# Autodesk Inventor assembly: 3_8 Shawny Lift 40t Idler
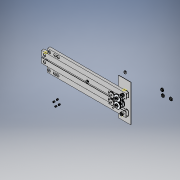
[picture p0: Inventor's stored thumbnail of the model, 180x180]
Saved by Autodesk Inventor 2018 (Build 220112000, 112)
## iProperties
Created: 2019-01-14
Part Number: 3_8 Shawny Lift 40t Idler
Document SubType Name: Assembly
Designer: Gabriel
Author: Gabriel
## Documents named in this file (10)
- C:\Users\Gabriel\Documents\3_8 Shawny Lift 40t Idler.iam
- C:\Users\Gabriel\Documents\8T spur gear 775.ipt
- C:\Users\Gabriel\Documents\36in Aluminum Channel OG.ipt
- C:\Users\Gabriel\Documents\Sanded Hex Rod.ipt
- C:\Users\Gabriel\Documents\Spacer 1 16 in.ipt
- C:\Users\Gabriel\Documents\Flanged bearing 3 8 in .ipt
- C:\Users\Gabriel\Documents\am-2300 Collar Clamp, 0.375'' Hex Bore, Aluminum REV2.iam
- C:\Users\Gabriel\Documents\50t 20dp 3 8 in gear.ipt
- C:\Users\Gabriel\Documents\40t_Aluminum_Spur_Gear_20_DP_3_8_Hex_Bore_217-2707.ipt
- C:\Users\Gabriel\Documents\Holding Plate.ipt
## Components (55 placed, 9 different names)
1. 8T spur gear 775:1
2. 8T spur gear 775:2
3. 8T spur gear 775:3
4. 8T spur gear 775:4
5. 36in Aluminum Channel OG:1 — Mate:1, Mate:2, Mate:3, Mate:4, Mate:5, Mate:6, Mate:7, Mate:8, Mate:78, Mate:79
6. Sanded Hex Rod:1 — Mate:25, Mate:29, Mate:30, Mate:35, Mate:36, Mate:59
7. 36in Aluminum Channel OG:2 — Mate:13, Mate:14, Mate:15, Mate:16, Mate:17, Mate:18, Mate:19, Mate:20, Mate:78, Mate:79
8. Sanded Hex Rod:4 — Mate:45, Mate:46, Mate:51, Mate:52, Mate:68, Mate:69
9. Flanged bearing 3 8 in :1 — Mate:13, Mate:14, Mate:31, Mate:59
10. Flanged bearing 3 8 in :2 — Mate:3, Mate:4, Mate:70, Mate:71, Mate:74
11. Flanged bearing 3 8 in :6 — Mate:1, Mate:2, Mate:47, Mate:68, Mate:69
12. Flanged bearing 3 8 in :7 — Mate:15, Mate:16, Mate:25, Mate:60, Mate:61, Mate:66
13. am-2300 Collar Clamp, 0.375'' Hex Bore, Aluminum REV2:1 [sub-assembly]
14. am-2300 Collar Clamp, 0.375'' Hex Bore, Aluminum REV2:2 [sub-assembly]
15. am-2300 Collar Clamp, 0.375'' Hex Bore, Aluminum REV2:3 [sub-assembly]
16. am-2300 Collar Clamp, 0.375'' Hex Bore, Aluminum REV2:5 [sub-assembly]
17. am-2300 Collar Clamp, 0.375'' Hex Bore, Aluminum REV2:7 [sub-assembly]
18. am-2300 Collar Clamp, 0.375'' Hex Bore, Aluminum REV2:8 [sub-assembly]
19. Spacer 1 16 in:3 — Mate:72, Mate:73, Mate:74, Mate:77
20. Spacer 1 16 in:4 — Mate:64, Mate:65, Mate:66, Mate:67
21. Spacer 1 16 in:5 — Mate:29, Mate:30, Mate:31, Mate:37
22. Spacer 1 16 in:6 — Mate:48, Mate:49, Mate:50, Mate:56
23. Spacer 1 16 in:7 — Mate:32, Mate:33, Mate:34, Mate:40
24. Spacer 1 16 in:8 — Mate:45, Mate:46, Mate:47, Mate:53
25. 50t 20dp 3 8 in gear:1 — Mate:35, Mate:36, Mate:37
26. 50t 20dp 3 8 in gear:4 — Mate:51, Mate:52, Mate:53
27. 50t 20dp 3 8 in gear:5 — Mate:75, Mate:76, Mate:77
28. 50t 20dp 3 8 in gear:7 — Mate:62, Mate:63, Mate:67
29. Flanged bearing 3 8 in :8 — Mate:19, Mate:20, Mate:27, Mate:28
30. Flanged bearing 3 8 in :11 — Mate:7, Mate:8, Mate:43, Mate:44
31. Flanged bearing 3 8 in :13 — Mate:17, Mate:18, Mate:34
32. Flanged bearing 3 8 in :15 — Mate:5, Mate:6, Mate:50
33. Sanded Hex Rod:5 — Mate:43, Mate:44, Mate:48, Mate:49, Mate:54, Mate:55
34. Sanded Hex Rod:8 — Mate:27, Mate:28, Mate:32, Mate:33, Mate:38, Mate:39
35. 40t_Aluminum_Spur_Gear_20_DP_3_8_Hex_Bore_217-2707:1 — Mate:38, Mate:39, Mate:40
36. 40t_Aluminum_Spur_Gear_20_DP_3_8_Hex_Bore_217-2707:2 — Mate:54, Mate:55, Mate:56
37. Sanded Hex Rod:9 — Mate:60, Mate:61, Mate:62, Mate:63, Mate:64, Mate:65
38. Sanded Hex Rod:10 — Mate:70, Mate:71, Mate:72, Mate:73, Mate:75, Mate:76
39. 36in Aluminum Channel OG:3 — Mate:89, Mate:90
40. 36in Aluminum Channel OG:4
41. Holding Plate:1 — Mate:80, Mate:81, Mate:82, Mate:83, Mate:84, Mate:85, Mate:86, Mate:87
42. Holding Plate:2 — Mate:94, Mate:95, Mate:96, Mate:97, Mate:98, Mate:99, Mate:100, Mate:101
43. Flanged bearing 3 8 in :16 — Mate:80, Mate:84
44. Flanged bearing 3 8 in :17 — Mate:81, Mate:85
45. Flanged bearing 3 8 in :18 — Mate:83, Mate:86
46. Flanged bearing 3 8 in :19 — Mate:82, Mate:87
47. Flanged bearing 3 8 in :20 — Mate:95, Mate:100
48. Flanged bearing 3 8 in :21 — Mate:97, Mate:98
49. Flanged bearing 3 8 in :22 — Mate:94, Mate:101
50. Flanged bearing 3 8 in :23 — Mate:96, Mate:99
51. Flanged bearing 3 8 in :24 — Mate:89, Mate:90, Mate:91, Mate:92
52. Flanged bearing 3 8 in :25
53. Flanged bearing 3 8 in :26
54. Flanged bearing 3 8 in :27
55. Sanded Hex Rod:11 — Mate:91, Mate:92
## Relationships (86: Mate 86)
- Mate:1: 36in Aluminum Channel OG:1 ↔ Flanged bearing 3 8 in :6
- Mate:2: 36in Aluminum Channel OG:1 ↔ Flanged bearing 3 8 in :6
- Mate:3: 36in Aluminum Channel OG:1 ↔ Flanged bearing 3 8 in :2
- Mate:4: 36in Aluminum Channel OG:1 ↔ Flanged bearing 3 8 in :2
- Mate:5: 36in Aluminum Channel OG:1 ↔ Flanged bearing 3 8 in :15
- Mate:6: 36in Aluminum Channel OG:1 ↔ Flanged bearing 3 8 in :15
- Mate:7: 36in Aluminum Channel OG:1 ↔ Flanged bearing 3 8 in :11
- Mate:8: 36in Aluminum Channel OG:1 ↔ Flanged bearing 3 8 in :11
- Mate:13: 36in Aluminum Channel OG:2 ↔ Flanged bearing 3 8 in :1
- Mate:14: 36in Aluminum Channel OG:2 ↔ Flanged bearing 3 8 in :1
- Mate:15: 36in Aluminum Channel OG:2 ↔ Flanged bearing 3 8 in :7
- Mate:16: 36in Aluminum Channel OG:2 ↔ Flanged bearing 3 8 in :7
- Mate:17: 36in Aluminum Channel OG:2 ↔ Flanged bearing 3 8 in :13
- Mate:18: 36in Aluminum Channel OG:2 ↔ Flanged bearing 3 8 in :13
- Mate:19: 36in Aluminum Channel OG:2 ↔ Flanged bearing 3 8 in :8
- Mate:20: 36in Aluminum Channel OG:2 ↔ Flanged bearing 3 8 in :8
- Mate:25: Sanded Hex Rod:1 ↔ Flanged bearing 3 8 in :7
- Mate:27: Flanged bearing 3 8 in :8 ↔ Sanded Hex Rod:8
- Mate:28: Flanged bearing 3 8 in :8 ↔ Sanded Hex Rod:8
- Mate:29: Sanded Hex Rod:1 ↔ Spacer 1 16 in:5
- Mate:30: Sanded Hex Rod:1 ↔ Spacer 1 16 in:5
- Mate:31: Flanged bearing 3 8 in :1 ↔ Spacer 1 16 in:5
- Mate:32: Spacer 1 16 in:7 ↔ Sanded Hex Rod:8
- Mate:33: Spacer 1 16 in:7 ↔ Sanded Hex Rod:8
- Mate:34: Spacer 1 16 in:7 ↔ Flanged bearing 3 8 in :13
- Mate:35: Sanded Hex Rod:1 ↔ 50t 20dp 3 8 in gear:1
- Mate:36: Sanded Hex Rod:1 ↔ 50t 20dp 3 8 in gear:1
- Mate:37: Spacer 1 16 in:5 ↔ 50t 20dp 3 8 in gear:1
- Mate:38: Sanded Hex Rod:8 ↔ 40t_Aluminum_Spur_Gear_20_DP_3_8_Hex_Bore_217-2707:1
- Mate:39: Sanded Hex Rod:8 ↔ 40t_Aluminum_Spur_Gear_20_DP_3_8_Hex_Bore_217-2707:1
- Mate:40: Spacer 1 16 in:7 ↔ 40t_Aluminum_Spur_Gear_20_DP_3_8_Hex_Bore_217-2707:1
- Mate:43: Flanged bearing 3 8 in :11 ↔ Sanded Hex Rod:5
- Mate:44: Flanged bearing 3 8 in :11 ↔ Sanded Hex Rod:5
- Mate:45: Sanded Hex Rod:4 ↔ Spacer 1 16 in:8
- Mate:46: Sanded Hex Rod:4 ↔ Spacer 1 16 in:8
- Mate:47: Flanged bearing 3 8 in :6 ↔ Spacer 1 16 in:8
- Mate:48: Spacer 1 16 in:6 ↔ Sanded Hex Rod:5
- Mate:49: Spacer 1 16 in:6 ↔ Sanded Hex Rod:5
- Mate:50: Spacer 1 16 in:6 ↔ Flanged bearing 3 8 in :15
- Mate:51: Sanded Hex Rod:4 ↔ 50t 20dp 3 8 in gear:4
- Mate:52: Sanded Hex Rod:4 ↔ 50t 20dp 3 8 in gear:4
- Mate:53: Spacer 1 16 in:8 ↔ 50t 20dp 3 8 in gear:4
- Mate:54: Sanded Hex Rod:5 ↔ 40t_Aluminum_Spur_Gear_20_DP_3_8_Hex_Bore_217-2707:2
- Mate:55: Sanded Hex Rod:5 ↔ 40t_Aluminum_Spur_Gear_20_DP_3_8_Hex_Bore_217-2707:2
- Mate:56: Spacer 1 16 in:6 ↔ 40t_Aluminum_Spur_Gear_20_DP_3_8_Hex_Bore_217-2707:2
- Mate:59: Sanded Hex Rod:1 ↔ Flanged bearing 3 8 in :1
- Mate:60: Flanged bearing 3 8 in :7 ↔ Sanded Hex Rod:9
- Mate:61: Flanged bearing 3 8 in :7 ↔ Sanded Hex Rod:9
- Mate:62: 50t 20dp 3 8 in gear:7 ↔ Sanded Hex Rod:9
- Mate:63: 50t 20dp 3 8 in gear:7 ↔ Sanded Hex Rod:9
- Mate:64: Spacer 1 16 in:4 ↔ Sanded Hex Rod:9
- Mate:65: Spacer 1 16 in:4 ↔ Sanded Hex Rod:9
- Mate:66: Flanged bearing 3 8 in :7 ↔ Spacer 1 16 in:4
- Mate:67: Spacer 1 16 in:4 ↔ 50t 20dp 3 8 in gear:7
- Mate:68: Sanded Hex Rod:4 ↔ Flanged bearing 3 8 in :6
- Mate:69: Sanded Hex Rod:4 ↔ Flanged bearing 3 8 in :6
- Mate:70: Flanged bearing 3 8 in :2 ↔ Sanded Hex Rod:10
- Mate:71: Flanged bearing 3 8 in :2 ↔ Sanded Hex Rod:10
- Mate:72: Spacer 1 16 in:3 ↔ Sanded Hex Rod:10
- Mate:73: Spacer 1 16 in:3 ↔ Sanded Hex Rod:10
- Mate:74: Flanged bearing 3 8 in :2 ↔ Spacer 1 16 in:3
- Mate:75: 50t 20dp 3 8 in gear:5 ↔ Sanded Hex Rod:10
- Mate:76: 50t 20dp 3 8 in gear:5 ↔ Sanded Hex Rod:10
- Mate:77: Spacer 1 16 in:3 ↔ 50t 20dp 3 8 in gear:5
- Mate:78 (12.7 mm): 36in Aluminum Channel OG:1 ↔ 36in Aluminum Channel OG:2
- Mate:79 (12.7 mm): 36in Aluminum Channel OG:1 ↔ 36in Aluminum Channel OG:2
- Mate:80: Holding Plate:1 ↔ Flanged bearing 3 8 in :16
- Mate:81: Holding Plate:1 ↔ Flanged bearing 3 8 in :17
- Mate:82: Holding Plate:1 ↔ Flanged bearing 3 8 in :19
- Mate:83: Holding Plate:1 ↔ Flanged bearing 3 8 in :18
- Mate:84: Holding Plate:1 ↔ Flanged bearing 3 8 in :16
- Mate:85: Holding Plate:1 ↔ Flanged bearing 3 8 in :17
- Mate:86: Holding Plate:1 ↔ Flanged bearing 3 8 in :18
- Mate:87: Holding Plate:1 ↔ Flanged bearing 3 8 in :19
- Mate:89: 36in Aluminum Channel OG:3 ↔ Flanged bearing 3 8 in :24
- Mate:90: 36in Aluminum Channel OG:3 ↔ Flanged bearing 3 8 in :24
- Mate:91: Flanged bearing 3 8 in :24 ↔ Sanded Hex Rod:11
- Mate:92: Flanged bearing 3 8 in :24 ↔ Sanded Hex Rod:11
- Mate:94: Holding Plate:2 ↔ Flanged bearing 3 8 in :22
- Mate:95: Holding Plate:2 ↔ Flanged bearing 3 8 in :20
- Mate:96: Holding Plate:2 ↔ Flanged bearing 3 8 in :23
- Mate:97: Holding Plate:2 ↔ Flanged bearing 3 8 in :21
- Mate:98: Holding Plate:2 ↔ Flanged bearing 3 8 in :21
- Mate:99: Holding Plate:2 ↔ Flanged bearing 3 8 in :23
- Mate:100: Holding Plate:2 ↔ Flanged bearing 3 8 in :20
- Mate:101: Holding Plate:2 ↔ Flanged bearing 3 8 in :22
